# Autodesk Inventor assembly: tank_flipper_v2_assembly
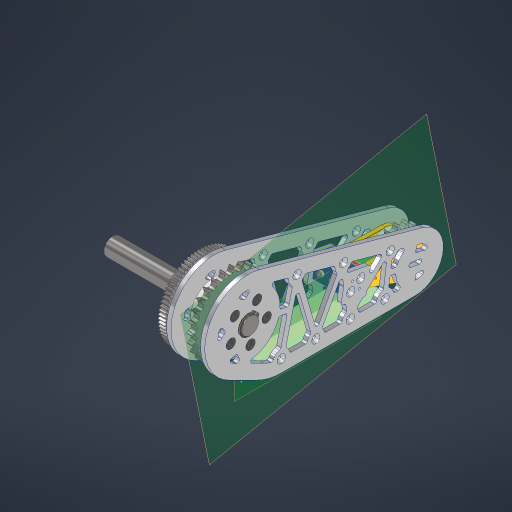
[picture p0: Inventor's stored thumbnail of the model, 512x512]
Saved by Autodesk Inventor 2023.2 (Build 272271030, 271C)
## iProperties
Created: 2023-04-05
Part Number: tank_flipper_v2_assembly
Document SubType Name: Assembly
Designer: ralph
Author: ralph
## Documents named in this file (13)
- C:\Users\ralph\OneDrive\Documents\GrabCAD\Robocup Rescue\Drive\v1\tank_flipper_v2_assembly.iam
- C:\Users\ralph\OneDrive\Documents\GrabCAD\Robocup Rescue\Drive\v1\TANK flipper\single tank.ipt
- C:\Users\ralph\OneDrive\Documents\GrabCAD\Robocup Rescue\Drive\v1\TANK flipper\panel bushing support.ipt
- C:\Users\ralph\OneDrive\Documents\GrabCAD\Robocup Rescue\Drive\v1\TANK flipper\2868T199_High-Load Oil-Embedded 863 Sleeve Bearing (1) v2(Mirror).ipt
- C:\Users\ralph\OneDrive\Documents\GrabCAD\Robocup Rescue\Drive\v1\TANK flipper\Drive Shaft.ipt
- C:\Users\ralph\OneDrive\Documents\GrabCAD\Robocup Rescue\Drive\v1\TANK flipper\98585A121_Heavy Duty External Retaining Ring v2(Mirror).ipt
- C:\Users\ralph\OneDrive\Documents\GrabCAD\Robocup Rescue\Drive\v1\TANK flipper\gearSpacer.ipt
- C:\Users\ralph\OneDrive\Documents\GrabCAD\Robocup Rescue\Drive\v1\TANK flipper\Spur Gear (74 teeth).ipt
- C:\Users\ralph\OneDrive\Documents\GrabCAD\Robocup Rescue\Drive\v1\TANK flipper\91259A167_Alloy Steel Shoulder Screw\91259A167_Alloy Steel Shoulder Screw.ipt
- C:\Users\ralph\OneDrive\Documents\GrabCAD\Robocup Rescue\Drive\v1\TANK flipper\27t track drive sprocket v25.iam
- C:\Users\ralph\OneDrive\Documents\GrabCAD\Robocup Rescue\Drive\v1\TANK flipper\flipper_tensioner.iam
- C:\Users\ralph\OneDrive\Documents\GrabCAD\Robocup Rescue\Drive\v1\TANK flipper\chain guide.ipt
- C:\Users\ralph\OneDrive\Documents\GrabCAD\Robocup Rescue\Drive\v1\TANK flipper\91263A553_Zinc-Plated Alloy Steel Hex Drive Flat Head Screw v1.ipt
## Components (26 placed, 12 different names)
1. single tank:1 — Rigid:2, Flush:1, Rigid:19, Rigid:20, Rigid:21, Rigid:22, Rotational:3
2. single tank:2 — Rigid:1, Rigid:8, Flush:1, Rigid:17, Rotational:2
3. panel bushing support:1 — Rigid:2, Rigid:4, Rigid:16
4. panel bushing support:2 — Rigid:1, Rigid:3, Rotational:1
5. 2868T199_High-Load Oil-Embedded 863 Sleeve Bearing (1) v2(Mirror):1 — Rigid:3
6. 2868T199_High-Load Oil-Embedded 863 Sleeve Bearing (1) v2(Mirror):2 — Rigid:4
7. Drive Shaft:1 — Rigid:5, Rotational:1, Rigid:14, Rigid:15, Rigid:16, Rigid:18
8. 98585A121_Heavy Duty External Retaining Ring v2(Mirror):1 — Rigid:5
9. gearSpacer:1 — Rigid:6, Rigid:8
10. Spur Gear (74 teeth):1 — Rigid:6, Rigid:7, Rigid:9, Rigid:10, Rigid:11, Rigid:12, Rigid:13
11. 2868T199_High-Load Oil-Embedded 863 Sleeve Bearing (1) v2(Mirror):3 — Rigid:7
12. 91259A167_Alloy Steel Shoulder Screw:1 — Rigid:9
13. 91259A167_Alloy Steel Shoulder Screw:2 — Rigid:13
14. 91259A167_Alloy Steel Shoulder Screw:3 — Rigid:12
15. 91259A167_Alloy Steel Shoulder Screw:4 — Rigid:11
16. 91259A167_Alloy Steel Shoulder Screw:5 — Rigid:10
17. 27t track drive sprocket v25:1 [sub-assembly] — Rigid:14
18. 98585A121_Heavy Duty External Retaining Ring v2(Mirror):2 — Rigid:15
19. 98585A121_Heavy Duty External Retaining Ring v2(Mirror):3 — Rigid:18
20. flipper_tensioner:1 [sub-assembly] — Rigid:17
21. chain guide:1 — Rotational:2
22. 91263A553_Zinc-Plated Alloy Steel Hex Drive Flat Head Screw v1:1 — Rotational:3
23. 91263A553_Zinc-Plated Alloy Steel Hex Drive Flat Head Screw v1:2 — Rigid:22
24. 91263A553_Zinc-Plated Alloy Steel Hex Drive Flat Head Screw v1:3 — Rigid:21
25. 91263A553_Zinc-Plated Alloy Steel Hex Drive Flat Head Screw v1:4 — Rigid:20
26. 91263A553_Zinc-Plated Alloy Steel Hex Drive Flat Head Screw v1:5 — Rigid:19
## Relationships (26: WeldJoint 22, RevoluteJoint 3, Flush 1)
- Rigid:1 [WeldJoint]: single tank:2 ↔ panel bushing support:2
- Rigid:2 [WeldJoint]: single tank:1 ↔ panel bushing support:1
- Rigid:3 [WeldJoint]: panel bushing support:2 ↔ 2868T199_High-Load Oil-Embedded 863 Sleeve Bearing (1) v2(Mirror):1
- Rigid:4 [WeldJoint]: panel bushing support:1 ↔ 2868T199_High-Load Oil-Embedded 863 Sleeve Bearing (1) v2(Mirror):2
- Rigid:5 [WeldJoint]: Drive Shaft:1 ↔ 98585A121_Heavy Duty External Retaining Ring v2(Mirror):1
- Rotational:1 [RevoluteJoint]: panel bushing support:2 ↔ Drive Shaft:1
- Rigid:6 [WeldJoint]: gearSpacer:1 ↔ Spur Gear (74 teeth):1
- Rigid:7 [WeldJoint]: Spur Gear (74 teeth):1 ↔ 2868T199_High-Load Oil-Embedded 863 Sleeve Bearing (1) v2(Mirror):3
- Rigid:8 [WeldJoint]: single tank:2 ↔ gearSpacer:1
- Rigid:9 [WeldJoint]: Spur Gear (74 teeth):1 ↔ 91259A167_Alloy Steel Shoulder Screw:1
- Rigid:10 [WeldJoint]: Spur Gear (74 teeth):1 ↔ 91259A167_Alloy Steel Shoulder Screw:5
- Rigid:11 [WeldJoint]: Spur Gear (74 teeth):1 ↔ 91259A167_Alloy Steel Shoulder Screw:4
- Rigid:12 [WeldJoint]: Spur Gear (74 teeth):1 ↔ 91259A167_Alloy Steel Shoulder Screw:3
- Rigid:13 [WeldJoint]: Spur Gear (74 teeth):1 ↔ 91259A167_Alloy Steel Shoulder Screw:2
- Rigid:14 [WeldJoint]: Drive Shaft:1 ↔ 27t track drive sprocket v25:1
- Rigid:15 [WeldJoint]: Drive Shaft:1 ↔ 98585A121_Heavy Duty External Retaining Ring v2(Mirror):2
- Rigid:16 [WeldJoint]: panel bushing support:1 ↔ Drive Shaft:1
- Flush:1: single tank:1 ↔ single tank:2
- Rigid:17 [WeldJoint]: single tank:2 ↔ flipper_tensioner:1
- Rotational:2 [RevoluteJoint]: single tank:2 ↔ chain guide:1
- Rigid:18 [WeldJoint]: Drive Shaft:1 ↔ 98585A121_Heavy Duty External Retaining Ring v2(Mirror):3
- Rigid:19 [WeldJoint]: single tank:1 ↔ 91263A553_Zinc-Plated Alloy Steel Hex Drive Flat Head Screw v1:5
- Rigid:20 [WeldJoint]: single tank:1 ↔ 91263A553_Zinc-Plated Alloy Steel Hex Drive Flat Head Screw v1:4
- Rigid:21 [WeldJoint]: single tank:1 ↔ 91263A553_Zinc-Plated Alloy Steel Hex Drive Flat Head Screw v1:3
- Rigid:22 [WeldJoint]: single tank:1 ↔ 91263A553_Zinc-Plated Alloy Steel Hex Drive Flat Head Screw v1:2
- Rotational:3 [RevoluteJoint]: single tank:1 ↔ 91263A553_Zinc-Plated Alloy Steel Hex Drive Flat Head Screw v1:1
